# Autodesk Inventor assembly: Assembly
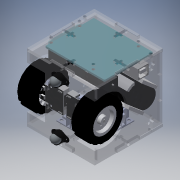
[picture p0: Inventor's stored thumbnail of the model, 180x180]
Saved by Autodesk Inventor 2016 (Build 200138000, 138)
## iProperties
Created: 2017-02-20
Part Number: Assembly
Document SubType Name: Assembly
Designer: jorge
Author: jorge
## Documents named in this file (20)
- C:\Users\jorge\Documents\Jorge P\Drive\Proyectos\Furo\CAD\Assembly.iam
- C:\Users\jorge\Documents\Jorge P\Drive\Proyectos\Furo\CAD\Base.ipt
- C:\Users\jorge\Documents\Jorge P\Drive\Proyectos\Furo\CAD\pared lateral.ipt
- C:\Users\jorge\Documents\Jorge P\Drive\Proyectos\Furo\CAD\pared frontal.ipt
- C:\Users\jorge\Documents\Jorge P\Drive\Proyectos\Furo\CAD\tapa superior.ipt
- C:\Users\jorge\Documents\Jorge P\Drive\Proyectos\Furo\CAD\Resources\Arduino\Arduino_Uno.ipt
- C:\Users\jorge\Documents\Jorge P\Drive\Proyectos\Furo\CAD\Resources\Pololu Caster Ball\Caster ball assembly.ipt
- C:\Users\jorge\Documents\Jorge P\Drive\Proyectos\Furo\CAD\Resources\bracket-pololu\Bracket Pololu.ipt
- C:\Users\jorge\Documents\Jorge P\Drive\Proyectos\Furo\CAD\Resources\dc-micromotor\micro motor pololu.ipt
- C:\Users\jorge\Documents\Jorge P\Drive\Proyectos\Furo\CAD\Resources\pololu-robot-wheel\pololu 1.65dia wheel.ipt
- C:\Users\jorge\Documents\Jorge P\Drive\Proyectos\Furo\CAD\Resources\arduino-driver-l298n\L298N.ipt
- C:\Users\jorge\Documents\Jorge P\Drive\Proyectos\Furo\CAD\Resources\esp8266-esp\ESP8266-ESP01.ipt
- C:\Users\jorge\Documents\Jorge P\Drive\Proyectos\Furo\CAD\Encoder.ipt
- C:\Users\jorge\Documents\Jorge P\Drive\Proyectos\Furo\CAD\pared ateral 2.ipt
- C:\Users\jorge\Documents\Jorge P\Drive\Proyectos\Furo\CAD\pared trasera.ipt
- C:\Users\jorge\Documents\Jorge P\Drive\Proyectos\Furo\CAD\bateria redonda.ipt
- C:\Users\jorge\Documents\Jorge P\Drive\Proyectos\Furo\CAD\soprte baterias.ipt
- C:\Users\jorge\Documents\Jorge P\Drive\Proyectos\Furo\CAD\soprte bateria parte 2.ipt
- C:\Users\jorge\Documents\Jorge P\Drive\Proyectos\Furo\CAD\soporte bateria parte 3.ipt
- C:\Users\jorge\Documents\Jorge P\Drive\Proyectos\Furo\CAD\soporte esp.ipt
## Components (24 placed, 19 different names)
1. Base:1 — Mate:4, Mate:5, Mate:6, Mate:9, Mate:16, Mate:17, Symmetry:1, Mate:43, Mate:49, Mate:50, Mate:51
2. pared lateral:2 — Mate:4, Mate:5, Mate:6, Flush:2, Flush:4, Mate:21, Mate:52, Flush:20, Mate:63
3. pared frontal:1 — Mate:9, Symmetry:1, Mate:60, Mate:61, Mate:62
4. tapa superior:1 — Flush:2, Flush:4, Angle:3, Mate:53, Flush:21, Flush:22, Mate:64, Flush:27
5. Caster ball assembly:1 — Mate:16, Mate:29, Tangent:1
6. Caster ball assembly:2 — Mate:17, Mate:21, Mate:30
7. L298N:1 — Mate:58, Mate:59, Flush:23, Mate:65
8. ESP8266-ESP01:1 — Mate:64, Mate:65, Mate:66
9. Encoder:1 — Mate:40, Mate:41, Angle:1, Mate:43, Flush:18, Flush:19, Symmetry:3
10. Bracket Pololu:2 — Mate:38, Mate:39, Flush:14, Mate:41, Angle:1, Flush:18
11. micro motor pololu:2 — Mate:38, Mate:39, Flush:14, Mate:40, Mate:42, Flush:15
12. pololu 1.65dia wheel:3 — Mate:42, Flush:15, Mate:49
13. Encoder:2 — Mate:50, Flush:19, Symmetry:3
14. Bracket Pololu:3 — Mate:59
15. micro motor pololu:3
16. pololu 1.65dia wheel:4 — Mate:51, Tangent:2
17. Arduino_Uno:1 — Mate:52, Flush:20, Mate:53
18. pared ateral 2:1 — Flush:21, Mate:58, Flush:23, Mate:66
19. pared trasera:1 — Flush:22, Flush:24
20. bateria redonda:1 — Mate:60, Mate:61, Mate:62, Mate:63, Flush:25, Flush:26
21. soprte baterias:1 — Flush:24
22. soprte bateria parte 2:1 — Flush:25
23. soporte bateria parte 3:1 — Flush:26
24. soporte esp:1 — Flush:27
## Relationships (58: Mate 34, Flush 16, Angle 4, Symmetry 2, Tangent 2)
- Mate:4: Base:1 ↔ pared lateral:2
- Mate:5: Base:1 ↔ pared lateral:2
- Mate:6: Base:1 ↔ pared lateral:2
- Mate:9: Base:1 ↔ pared frontal:1
- Flush:2: pared lateral:2 ↔ tapa superior:1
- Flush:4: pared lateral:2 ↔ tapa superior:1
- Mate:16: Base:1 ↔ Caster ball assembly:1
- Mate:17: Base:1 ↔ Caster ball assembly:2
- Mate:21 (-10 mm): pared lateral:2 ↔ Caster ball assembly:2
- Symmetry:1: Base:1 ↔ pared frontal:1
- Mate:29: Caster ball assembly:1
- Mate:30: Caster ball assembly:2
- Mate:38: Bracket Pololu:2 ↔ micro motor pololu:2
- Mate:39: Bracket Pololu:2 ↔ micro motor pololu:2
- Flush:14: Bracket Pololu:2 ↔ micro motor pololu:2
- Mate:40: Encoder:1 ↔ micro motor pololu:2
- Mate:41: Encoder:1 ↔ Bracket Pololu:2
- Angle:1 (0 deg): Encoder:1 ↔ Bracket Pololu:2
- Mate:42: micro motor pololu:2 ↔ pololu 1.65dia wheel:3
- Flush:15: micro motor pololu:2 ↔ pololu 1.65dia wheel:3
- Mate:43: Base:1 ↔ Encoder:1
- [Mate]: Bracket Pololu:3 ↔ micro motor pololu:3
- [Mate]: Bracket Pololu:3 ↔ micro motor pololu:3
- [Flush]: Bracket Pololu:3 ↔ micro motor pololu:3
- [Mate]: Encoder:2 ↔ micro motor pololu:3
- [Mate]: Encoder:2 ↔ Bracket Pololu:3
- [Angle] (0 deg): Encoder:2 ↔ Bracket Pololu:3
- [Mate]: micro motor pololu:3 ↔ pololu 1.65dia wheel:4
- [Flush]: micro motor pololu:3 ↔ pololu 1.65dia wheel:4
- Flush:18 (4.156 mm): Encoder:1 ↔ Bracket Pololu:2
- Mate:49 (3 mm): Base:1 ↔ pololu 1.65dia wheel:3
- Mate:50: Base:1 ↔ Encoder:2
- Mate:51 (3 mm): Base:1 ↔ pololu 1.65dia wheel:4
- Flush:19: Encoder:1 ↔ Encoder:2
- Symmetry:3: Encoder:1 ↔ Encoder:2
- Angle:3 (0 deg): tapa superior:1
- Tangent:1: Caster ball assembly:1
- Angle:4 (0 deg)
- Tangent:2: pololu 1.65dia wheel:4
- Mate:52 (2 mm): pared lateral:2 ↔ Arduino_Uno:1
- Flush:20: pared lateral:2 ↔ Arduino_Uno:1
- Mate:53 (1 mm): tapa superior:1 ↔ Arduino_Uno:1
- Flush:21: tapa superior:1 ↔ pared ateral 2:1
- Flush:22: tapa superior:1 ↔ pared trasera:1
- Mate:58 (1.5 mm): L298N:1 ↔ pared ateral 2:1
- Mate:59: L298N:1 ↔ Bracket Pololu:3
- Flush:23 (13 mm): L298N:1 ↔ pared ateral 2:1
- Mate:60 (-13.5 mm): pared frontal:1 ↔ bateria redonda:1
- Mate:61: pared frontal:1 ↔ bateria redonda:1
- Mate:62: pared frontal:1 ↔ bateria redonda:1
- Mate:63 (27 mm): pared lateral:2 ↔ bateria redonda:1
- Flush:24: pared trasera:1 ↔ soprte baterias:1
- Flush:25: bateria redonda:1 ↔ soprte bateria parte 2:1
- Flush:26: bateria redonda:1 ↔ soporte bateria parte 3:1
- Mate:64: tapa superior:1 ↔ ESP8266-ESP01:1
- Mate:65 (8 mm): L298N:1 ↔ ESP8266-ESP01:1
- Mate:66 (2 mm): ESP8266-ESP01:1 ↔ pared ateral 2:1
- Flush:27: tapa superior:1 ↔ soporte esp:1
## Named parameters: d71_d69 = 0 mm, d72_d62 = 0 mm, d73_d63 = 0 mm, d74_d64 = 0 mm, d75_d65 = 0 mm, d76_d66 = 0 mm, d77_d67 = 0 deg, d78_d68 = 0 mm
